# Autodesk Inventor assembly: Front Left Upper Arm Assembly
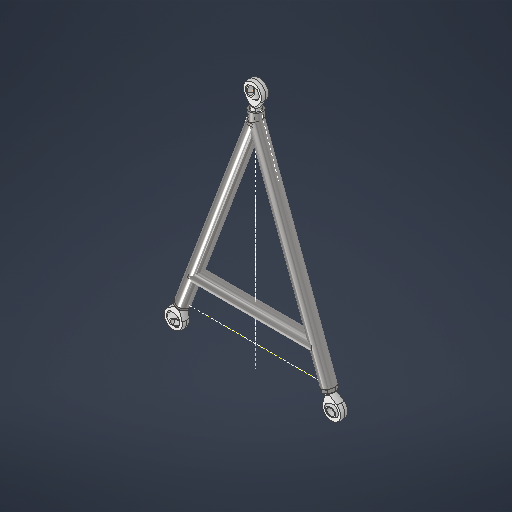
[picture p0: Inventor's stored thumbnail of the model, 512x512]
Saved by Autodesk Inventor 2026.1 (Build 301233000, 233)
## iProperties
Created: 2026-07-08
Part Number: Front Left Upper Arm Assembly
Document SubType Name: Assembly
Designer: share
_SolveAssemblyDoc: Frame Generator Solve Assembly
_Version: 15.0.0
Author: share
## iProperties of the stored document MemberDocs/xIow4bf5tKs1rnmvdSscz5bf5Xe
Created: 2026-07-08
Part Number: Front Left Upper Arm Assembly
Document SubType Name: Assembly
Designer: share
_SolveAssemblyDoc: Frame Generator Solve Assembly
_Version: 15.0.0
Author: share
## iProperties of the stored document MemberDocs/x3busjfcqDcewfwirL2nfthnpPh
_SolveAssemblyDoc: Frame Generator Solve Assembly
_Version: 15.0.0
Created: 2026-07-08
Part Number: Front Left Upper Arm Assembly
Document SubType Name: Assembly
Designer: share
Author: share
## iProperties of the stored document MemberDocs/xJhbfjznsAcrda2x4Ownp1f2uDd
Created: 2026-07-08
Part Number: Front Left Upper Arm Assembly
Document SubType Name: Assembly
Designer: share
_SolveAssemblyDoc: Frame Generator Solve Assembly
_Version: 15.0.0
Author: share
## iProperties of the stored document MemberDocs/xOvykjulhN0jdcosyVem1lpf5Qf
Created: 2026-07-08
Part Number: Front Left Upper Arm Assembly
Document SubType Name: Assembly
Designer: share
_SolveAssemblyDoc: Frame Generator Solve Assembly
_Version: 15.0.0
Author: share
## Documents named in this file (7)
- C:\Users\share\OneDrive\Documents\Personal Projects\GOGO Kart\CAD\GOGO_KART_FSAE\Suspension\Suspension Arms\Front Left\Front Left Lower Arm Assembly.iam
- C:\Users\share\OneDrive\Documents\Personal Projects\GOGO Kart\CAD\GOGO_KART_FSAE\Suspension\Suspension Arms\Arm_Outline_Sketch.ipt
- C:\Users\share\OneDrive\Documents\Personal Projects\GOGO Kart\CAD\GOGO_KART_FSAE\Suspension\Suspension Arms\Suspension Arm Assembly\Frame\Frame 1783539100150.iam
- C:\Users\share\OneDrive\Documents\Inventor\Content Center Files\R2026\en-US\ISO 8675(2)\ISO 8675 - M12 x 1.5 - ISO.ipt
- C:\Users\share\OneDrive\Documents\Personal Projects\GOGO Kart\CAD\GOGO_KART_FSAE\Rod Ends\5-8 Rod End\Suspension Rod Ends\Front Left\Lower\5-8 Rod End Assembly-Lower-FL-LF.iam
- C:\Users\share\OneDrive\Documents\Personal Projects\GOGO Kart\CAD\GOGO_KART_FSAE\Rod Ends\5-8 Rod End\Suspension Rod Ends\Front Left\Lower\5-8 Rod End Assembly-Lower-FL-LR.iam
- C:\Users\share\OneDrive\Documents\Personal Projects\GOGO Kart\CAD\GOGO_KART_FSAE\Rod Ends\5-8 Rod End\Suspension Rod Ends\Front Left\Lower\5-8 Rod End Assembly-Lower-FL-LOP.iam
## Components (8 placed, 6 different names)
1. Arm_Outline_Sketch:1 — Flush:1, Flush:2, Flush:3, Mate:1, Mate:2, Mate:3, Mate:4, Mate:5, Mate:6, Mate:7, Mate:8, Mate:9
2. Frame 1783539100150:1 [sub-assembly] — Insert:1, Insert:2, Insert:3
3. ISO 8675 M12 x 1.5:1 — Insert:1
4. ISO 8675 M12 x 1.5:2 — Insert:2
5. ISO 8675 M12 x 1.5:3 — Insert:3
6. 5-8 Rod End Assembly-Lower-FL-LF:1 [sub-assembly] — Mate:1, Mate:2, Mate:3
7. 5-8 Rod End Assembly-Lower-FL-LR:1 [sub-assembly] — Mate:4, Mate:5, Mate:9
8. 5-8 Rod End Assembly-Lower-FL-LOP:1 [sub-assembly] — Mate:6, Mate:7, Mate:8
## Relationships (15: Mate 9, Insert 3, Flush 3)
- Insert:1: Frame 1783539100150:1 ↔ ISO 8675 M12 x 1.5:1
- Insert:2: Frame 1783539100150:1 ↔ ISO 8675 M12 x 1.5:2
- Insert:3: Frame 1783539100150:1 ↔ ISO 8675 M12 x 1.5:3
- Flush:1: Arm_Outline_Sketch:1
- Flush:2: Arm_Outline_Sketch:1
- Flush:3 (-88.788 mm): Arm_Outline_Sketch:1
- Mate:1: Arm_Outline_Sketch:1 ↔ 5-8 Rod End Assembly-Lower-FL-LF:1
- Mate:2: Arm_Outline_Sketch:1 ↔ 5-8 Rod End Assembly-Lower-FL-LF:1
- Mate:3: Arm_Outline_Sketch:1 ↔ 5-8 Rod End Assembly-Lower-FL-LF:1
- Mate:4: Arm_Outline_Sketch:1 ↔ 5-8 Rod End Assembly-Lower-FL-LR:1
- Mate:5: Arm_Outline_Sketch:1 ↔ 5-8 Rod End Assembly-Lower-FL-LR:1
- Mate:6: Arm_Outline_Sketch:1 ↔ 5-8 Rod End Assembly-Lower-FL-LOP:1
- Mate:7: Arm_Outline_Sketch:1 ↔ 5-8 Rod End Assembly-Lower-FL-LOP:1
- Mate:8: Arm_Outline_Sketch:1 ↔ 5-8 Rod End Assembly-Lower-FL-LOP:1
- Mate:9: Arm_Outline_Sketch:1 ↔ 5-8 Rod End Assembly-Lower-FL-LR:1
